# Autodesk Inventor assembly: Backpack
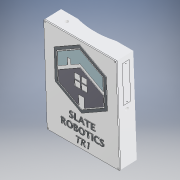
[picture p0: Inventor's stored thumbnail of the model, 180x180]
Saved by Autodesk Inventor 2017 SP1 (Build 210196100, 196)
## iProperties
Created: 2017-09-05
Part Number: Backpack
Document SubType Name: Assembly
Designer: Zach
Author: Zach
## Documents named in this file (7)
- C:\Users\Zach\Documents\GitHub\tr1\src\Body\Chest Assembly\Backpack Assembly\Backpack.iam
- C:\Users\Zach\Documents\GitHub\tr1\src\Body\Chest Assembly\Backpack Assembly\BP001b.ipt
- C:\Users\Zach\Documents\GitHub\tr1\src\Body\Chest Assembly\Backpack Assembly\BP002b.ipt
- C:\Users\Zach\Documents\GitHub\tr1\src\Body\Chest Assembly\Backpack Assembly\BP003.ipt
- C:\Users\Zach\Documents\GitHub\tr1\src\Body\Chest Assembly\Backpack Assembly\BP004.ipt
- C:\Users\Zach\Documents\GitHub\tr1\src\Body\Chest Assembly\Backpack Assembly\BP005.ipt
- C:\Users\Zach\Documents\GitHub\tr1\src\Body\Chest Assembly\Backpack Assembly\BP006.ipt
## Components (7 placed, 6 different names)
1. BP001b:1 — Mate:1, Mate:2, Mate:3, Mate:5, Mate:6, Mate:7, Mate:8, Mate:9, Mate:11, Mate:13, Mate:14, Mate:15, Mate:16, Mate:17, Mate:18, Mate:19, Mate:20, Mate:21
2. BP002b:1 — Mate:1, Mate:2, Mate:3
3. BP003:1 — Mate:14, Mate:15, Mate:16
4. BP004:1 — Mate:5, Mate:6, Mate:7
5. BP005:1 — Mate:8, Mate:9, Mate:20
6. BP006:1 — Mate:11, Mate:13, Mate:21
7. BP003:2 — Mate:17, Mate:18, Mate:19
## Relationships (18: Mate 18)
- Mate:1: BP001b:1 ↔ BP002b:1
- Mate:2: BP001b:1 ↔ BP002b:1
- Mate:3: BP001b:1 ↔ BP002b:1
- Mate:5: BP001b:1 ↔ BP004:1
- Mate:6: BP001b:1 ↔ BP004:1
- Mate:7: BP001b:1 ↔ BP004:1
- Mate:8: BP001b:1 ↔ BP005:1
- Mate:9: BP001b:1 ↔ BP005:1
- Mate:11: BP001b:1 ↔ BP006:1
- Mate:13: BP001b:1 ↔ BP006:1
- Mate:14: BP001b:1 ↔ BP003:1
- Mate:15: BP001b:1 ↔ BP003:1
- Mate:16: BP001b:1 ↔ BP003:1
- Mate:17: BP001b:1 ↔ BP003:2
- Mate:18: BP001b:1 ↔ BP003:2
- Mate:19: BP001b:1 ↔ BP003:2
- Mate:20: BP001b:1 ↔ BP005:1
- Mate:21: BP001b:1 ↔ BP006:1
